# Autodesk Inventor assembly: Z Axis_MIR
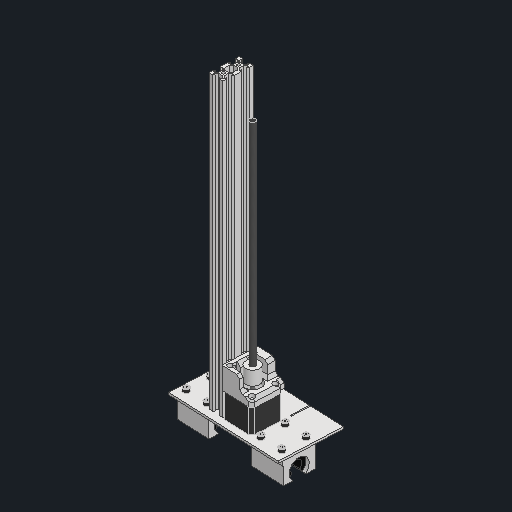
[picture p0: Inventor's stored thumbnail of the model, 512x512]
Saved by Autodesk Inventor 2025.1 (Build 291241000, 241)
## iProperties
Created: 2025-01-21
Part Number: Z Axis_MIR
Document SubType Name: Assembly
Designer: jerem
Author: jerem
## Documents named in this file (10)
- C:\Users\jerem\Documents\GitHub\Perovskite-Automated-Synthesis-System\CAD\Gantry\Z Axis\Z Axis_MIR.iam
- C:\Users\jerem\Documents\GitHub\Perovskite-Automated-Synthesis-System\CAD\Non 3D Printed Parts\Extrusion\V Extrustion 40x400mm.ipt
- C:\Users\jerem\Documents\GitHub\Perovskite-Automated-Synthesis-System\CAD\Non 3D Printed Parts\Screws\M5x12.ipt
- C:\Users\jerem\Documents\GitHub\Perovskite-Automated-Synthesis-System\CAD\Non 3D Printed Parts\Motors and Servos\NEMA17 Stepper Motor.ipt
- C:\Users\jerem\Documents\GitHub\Perovskite-Automated-Synthesis-System\CAD\Non 3D Printed Parts\Threaded Rod 300mm.ipt
- C:\Users\jerem\Documents\GitHub\Perovskite-Automated-Synthesis-System\CAD\Non 3D Printed Parts\Rod Coupler.ipt
- C:\Users\jerem\Documents\GitHub\Perovskite-Automated-Synthesis-System\CAD\Non 3D Printed Parts\Nuts\M4 T-Slot Nut.ipt
- C:\Users\jerem\Documents\GitHub\Perovskite-Automated-Synthesis-System\CAD\Gantry\Z Axis\Z Axis Motor Mount.ipt
- C:\Users\jerem\Documents\GitHub\Perovskite-Automated-Synthesis-System\CAD\Non 3D Printed Parts\Linear Rails\Linear Rail Slider Block.ipt
- C:\Users\jerem\Documents\GitHub\Perovskite-Automated-Synthesis-System\CAD\Non 3D Printed Parts\X Axis Base Plate Accurate_MIR.ipt
## Components (18 placed, 9 different names)
1. V Extrustion 40x400mm:1 — Mate:13, Mate:14, Mate:28, Mate:31, Mate:32
2. M5x12:1 — Mate:8, Mate:19
3. M5x12:2 — Mate:9, Mate:20
4. M5x12:3 — Mate:6, Mate:39, Mate:40
5. M5x12:4 — Mate:5, Mate:37
6. M5x12:5 — Mate:22, Mate:23
7. M5x12:6 — Mate:10, Mate:21
8. NEMA17 Stepper Motor:1 — Mate:15, Mate:16, Mate:17, Mate:18, Mate:24, Mate:25, Mate:31
9. Threaded Rod 300mm:1 — Mate:24, Mate:25, Mate:26, Mate:27
10. Rod Coupler:1 — Mate:26, Mate:27
11. M4 T-Slot Nut:1 — Mate:29, Mate:34, Angle:2
12. M4 T-Slot Nut:2 — Mate:30, Mate:33, Angle:1
13. Z Axis Motor Mount:1 — Mate:15, Mate:16, Mate:17, Mate:29, Mate:30, Mate:32, Mate:33, Mate:34, Angle:1, Angle:2
14. Linear Rail Slider Block:1 — Mate:1, Mate:11, Mate:12
15. X Axis Base Plate Accurate_MIR:1 — Mate:1, Mate:2, Mate:3, Mate:4, Mate:5, Mate:6, Mate:7, Mate:8, Mate:9, Mate:10, Mate:11, Mate:12, Mate:13, Mate:14, Mate:18, Mate:19, Mate:20, Mate:21, Mate:22, Mate:23, Mate:28, Mate:35, Mate:36, Mate:37, Mate:38, Mate:39
16. Linear Rail Slider Block:2 — Mate:2, Mate:3, Mate:40
17. M5x12:7 — Mate:4, Mate:35, Mate:36
18. M5x12:8 — Mate:7, Mate:38
## Relationships (42: Mate 40, Angle 2)
- Mate:1: Linear Rail Slider Block:1 ↔ X Axis Base Plate Accurate_MIR:1
- Mate:2: X Axis Base Plate Accurate_MIR:1 ↔ Linear Rail Slider Block:2
- Mate:3: X Axis Base Plate Accurate_MIR:1 ↔ Linear Rail Slider Block:2
- Mate:4: X Axis Base Plate Accurate_MIR:1 ↔ M5x12:7
- Mate:5: M5x12:4 ↔ X Axis Base Plate Accurate_MIR:1
- Mate:6: M5x12:3 ↔ X Axis Base Plate Accurate_MIR:1
- Mate:7: X Axis Base Plate Accurate_MIR:1 ↔ M5x12:8
- Mate:8: M5x12:1 ↔ X Axis Base Plate Accurate_MIR:1
- Mate:9: M5x12:2 ↔ X Axis Base Plate Accurate_MIR:1
- Mate:10: M5x12:6 ↔ X Axis Base Plate Accurate_MIR:1
- Mate:11: Linear Rail Slider Block:1 ↔ X Axis Base Plate Accurate_MIR:1
- Mate:12: Linear Rail Slider Block:1 ↔ X Axis Base Plate Accurate_MIR:1
- Mate:13: V Extrustion 40x400mm:1 ↔ X Axis Base Plate Accurate_MIR:1
- Mate:14: V Extrustion 40x400mm:1 ↔ X Axis Base Plate Accurate_MIR:1
- Mate:15: NEMA17 Stepper Motor:1 ↔ Z Axis Motor Mount:1
- Mate:16: NEMA17 Stepper Motor:1 ↔ Z Axis Motor Mount:1
- Mate:17: NEMA17 Stepper Motor:1 ↔ Z Axis Motor Mount:1
- Mate:18: NEMA17 Stepper Motor:1 ↔ X Axis Base Plate Accurate_MIR:1
- Mate:19: M5x12:1 ↔ X Axis Base Plate Accurate_MIR:1
- Mate:20: M5x12:2 ↔ X Axis Base Plate Accurate_MIR:1
- Mate:21: M5x12:6 ↔ X Axis Base Plate Accurate_MIR:1
- Mate:22: M5x12:5 ↔ X Axis Base Plate Accurate_MIR:1
- Mate:23: M5x12:5 ↔ X Axis Base Plate Accurate_MIR:1
- Mate:24: NEMA17 Stepper Motor:1 ↔ Threaded Rod 300mm:1
- Mate:25: NEMA17 Stepper Motor:1 ↔ Threaded Rod 300mm:1
- Mate:26: Threaded Rod 300mm:1 ↔ Rod Coupler:1
- Mate:27: Threaded Rod 300mm:1 ↔ Rod Coupler:1
- Mate:28: V Extrustion 40x400mm:1 ↔ X Axis Base Plate Accurate_MIR:1
- Mate:29: M4 T-Slot Nut:1 ↔ Z Axis Motor Mount:1
- Mate:30: M4 T-Slot Nut:2 ↔ Z Axis Motor Mount:1
- Mate:31: V Extrustion 40x400mm:1 ↔ NEMA17 Stepper Motor:1
- Mate:32: V Extrustion 40x400mm:1 ↔ Z Axis Motor Mount:1
- Mate:33: M4 T-Slot Nut:2 ↔ Z Axis Motor Mount:1
- Mate:34: M4 T-Slot Nut:1 ↔ Z Axis Motor Mount:1
- Angle:1 (0 deg): M4 T-Slot Nut:2 ↔ Z Axis Motor Mount:1
- Angle:2 (0 deg): M4 T-Slot Nut:1 ↔ Z Axis Motor Mount:1
- Mate:35: X Axis Base Plate Accurate_MIR:1 ↔ M5x12:7
- Mate:36: X Axis Base Plate Accurate_MIR:1 ↔ M5x12:7
- Mate:37: M5x12:4 ↔ X Axis Base Plate Accurate_MIR:1
- Mate:38: X Axis Base Plate Accurate_MIR:1 ↔ M5x12:8
- Mate:39: M5x12:3 ↔ X Axis Base Plate Accurate_MIR:1
- Mate:40: M5x12:3 ↔ Linear Rail Slider Block:2
